# Autodesk Inventor assembly: assembly_support
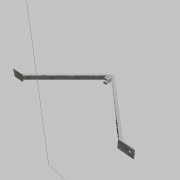
[picture p0: Inventor's stored thumbnail of the model, 180x180]
Saved by Autodesk Inventor 2021 (Build 250183000, 183)
## iProperties
Created: 2021-05-11
Part Number: assembly_support
Document SubType Name: Assembly
Designer: Watchdog
Author: Watchdog
## Documents named in this file (3)
- C:\Users\Watchdog\OneDrive - Flinders\Advn Mech Design Shared\6_Development\2_Design\inventor\support\assembly_support.iam
- C:\Users\Watchdog\OneDrive - Flinders\Advn Mech Design Shared\6_Development\2_Design\inventor\support\support_weldAssembly.iam
- C:\Users\Watchdog\OneDrive - Flinders\Advn Mech Design Shared\6_Development\2_Design\inventor\support\support_sandwichPlate.ipt
## Components (3 placed, 2 different names)
1. support_weldAssembly:1 [sub-assembly] — Mate:1, Mate:2, Mate:3, Flush:1, Mate:6, Mate:7
2. support_weldAssembly:2 [sub-assembly] — Mate:5, Flush:2, Mate:8
3. support_sandwichPlate:1 — Flush:1, Mate:5, Flush:2, Mate:6, Mate:7, Mate:8
## Relationships (9: Mate 7, Flush 2)
- Mate:1: support_weldAssembly:1
- Mate:2: support_weldAssembly:1
- Mate:3: support_weldAssembly:1
- Flush:1: support_weldAssembly:1 ↔ support_sandwichPlate:1
- Mate:5: support_weldAssembly:2 ↔ support_sandwichPlate:1
- Flush:2: support_weldAssembly:2 ↔ support_sandwichPlate:1
- Mate:6: support_weldAssembly:1 ↔ support_sandwichPlate:1
- Mate:7: support_weldAssembly:1 ↔ support_sandwichPlate:1
- Mate:8: support_weldAssembly:2 ↔ support_sandwichPlate:1
